# Autodesk Inventor assembly: carrier
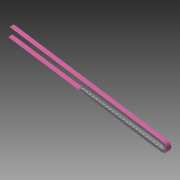
[picture p0: Inventor's stored thumbnail of the model, 180x180]
Saved by Autodesk Inventor 2013 (Build 170138000, 138)
## iProperties
Created: 2013-01-17
Part Number: carrier
Document SubType Name: Assembly
Designer: istvan.burbank
Author: istvan.burbank
## Documents named in this file (5)
- E:\GitHub\Crown-Fire\CAD\Electronics\carrier\carrier.iam
- E:\GitHub\Crown-Fire\CAD\Electronics\carrier\carrier12.iam
- E:\GitHub\Crown-Fire\CAD\Electronics\carrier\guide.ipt
- E:\GitHub\Crown-Fire\CAD\Electronics\carrier\carrierSegment.ipt
- E:\GitHub\Crown-Fire\CAD\Electronics\carrier\carrier20.iam
## Components (5 placed, 4 different names)
1. carrierSegment:1 — Mate:1, Mate:2, Flush:1, Mate:3
2. carrier12:1 [sub-assembly] — Mate:1, Mate:2, Mate:11, Mate:12, Transitional:1, Transitional:2, Transitional:3, Transitional:4, Transitional:5, Transitional:6, Transitional:7, Transitional:8, Transitional:9, Transitional:10, Transitional:11
3. carrier20:4 [sub-assembly] — Mate:11, Mate:12, Transitional:12, Transitional:13, Transitional:14, Transitional:15, Transitional:16, Transitional:17, Transitional:18, Transitional:20, Transitional:21, Transitional:22, Transitional:23, Transitional:24, Transitional:25, Transitional:26, Transitional:27, Transitional:28, Transitional:29, Mate:14, Transitional:30, Transitional:31, Transitional:32, Mate:16
4. carrier20:5 [sub-assembly] — Mate:14, Mate:16, Transitional:33, Transitional:34, Transitional:35, Transitional:36, Transitional:37, Transitional:38, Transitional:39, Transitional:40, Transitional:41, Transitional:42, Transitional:43, Transitional:44, Transitional:45, Transitional:46, Mate:17, Transitional:47, Transitional:48, Transitional:49, Transitional:50, Transitional:51, Transitional:52
5. guide:1 — Flush:1, Mate:3, Transitional:1, Transitional:2, Transitional:3, Transitional:4, Transitional:5, Transitional:6, Transitional:7, Transitional:8, Transitional:9, Transitional:10, Transitional:11, Transitional:12, Transitional:13, Transitional:14, Transitional:15, Transitional:16, Transitional:17, Transitional:18, Transitional:20, Transitional:21, Transitional:22, Transitional:23, Transitional:24, Transitional:25, Transitional:26, Transitional:27, Transitional:28, Transitional:29, Transitional:30, Transitional:31, Transitional:32, Transitional:33, Transitional:34, Transitional:35, Transitional:36, Transitional:37, Transitional:38, Transitional:39, Transitional:40, Transitional:41, Transitional:42, Transitional:43, Transitional:44, Transitional:45, Transitional:46, Mate:17, Transitional:47, Transitional:48, Transitional:49, Transitional:50, Transitional:51, Transitional:52
## Relationships (60: Transitional 51, Mate 8, Flush 1)
- Mate:1: carrierSegment:1 ↔ carrier12:1
- Mate:2: carrierSegment:1 ↔ carrier12:1
- Flush:1: carrierSegment:1 ↔ guide:1
- Mate:3: carrierSegment:1 ↔ guide:1
- Mate:11: carrier12:1 ↔ carrier20:4
- Mate:12: carrier12:1 ↔ carrier20:4
- Transitional:1: carrier12:1 ↔ guide:1
- Transitional:2: carrier12:1 ↔ guide:1
- Transitional:3: carrier12:1 ↔ guide:1
- Transitional:4: carrier12:1 ↔ guide:1
- Transitional:5: carrier12:1 ↔ guide:1
- Transitional:6: carrier12:1 ↔ guide:1
- Transitional:7: carrier12:1 ↔ guide:1
- Transitional:8: carrier12:1 ↔ guide:1
- Transitional:9: carrier12:1 ↔ guide:1
- Transitional:10: carrier12:1 ↔ guide:1
- Transitional:11: carrier12:1 ↔ guide:1
- Transitional:12: carrier20:4 ↔ guide:1
- Transitional:13: carrier20:4 ↔ guide:1
- Transitional:14: carrier20:4 ↔ guide:1
- Transitional:15: carrier20:4 ↔ guide:1
- Transitional:16: carrier20:4 ↔ guide:1
- Transitional:17: carrier20:4 ↔ guide:1
- Transitional:18: carrier20:4 ↔ guide:1
- Transitional:20: carrier20:4 ↔ guide:1
- Transitional:21: carrier20:4 ↔ guide:1
- Transitional:22: carrier20:4 ↔ guide:1
- Transitional:23: carrier20:4 ↔ guide:1
- Transitional:24: carrier20:4 ↔ guide:1
- Transitional:25: carrier20:4 ↔ guide:1
- Transitional:26: carrier20:4 ↔ guide:1
- Transitional:27: carrier20:4 ↔ guide:1
- Transitional:28: carrier20:4 ↔ guide:1
- Transitional:29: carrier20:4 ↔ guide:1
- Mate:14: carrier20:4 ↔ carrier20:5
- Transitional:30: carrier20:4 ↔ guide:1
- Transitional:31: carrier20:4 ↔ guide:1
- Transitional:32: carrier20:4 ↔ guide:1
- Mate:16: carrier20:4 ↔ carrier20:5
- Transitional:33: carrier20:5 ↔ guide:1
- Transitional:34: carrier20:5 ↔ guide:1
- Transitional:35: carrier20:5 ↔ guide:1
- Transitional:36: carrier20:5 ↔ guide:1
- Transitional:37: carrier20:5 ↔ guide:1
- Transitional:38: carrier20:5 ↔ guide:1
- Transitional:39: carrier20:5 ↔ guide:1
- Transitional:40: carrier20:5 ↔ guide:1
- Transitional:41: carrier20:5 ↔ guide:1
- Transitional:42: carrier20:5 ↔ guide:1
- Transitional:43: carrier20:5 ↔ guide:1
- Transitional:44: carrier20:5 ↔ guide:1
- Transitional:45: carrier20:5 ↔ guide:1
- Transitional:46: carrier20:5 ↔ guide:1
- Mate:17: carrier20:5 ↔ guide:1
- Transitional:47: carrier20:5 ↔ guide:1
- Transitional:48: carrier20:5 ↔ guide:1
- Transitional:49: carrier20:5 ↔ guide:1
- Transitional:50: carrier20:5 ↔ guide:1
- Transitional:51: carrier20:5 ↔ guide:1
- Transitional:52: carrier20:5 ↔ guide:1
